# Autodesk Inventor assembly: caseBody_basePlate
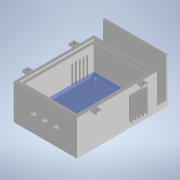
[picture p0: Inventor's stored thumbnail of the model, 180x180]
Saved by Autodesk Inventor 2022.6 (Build 266554010, 554A)
## iProperties
Created: 2025-03-20
Part Number: caseBody_basePlate
Document SubType Name: Assembly
Designer: khinm
Author: khinm
## Documents named in this file (3)
- C:\Users\khinm\Downloads\CAD\toolkit_controllerCaseDesign\caseBody_basePlate.iam
- C:\Users\khinm\Downloads\CAD\basePlate.ipt
- C:\Users\khinm\Downloads\CAD\caseBody.ipt
## Components (2 placed, 2 different names)
1. basePlate:1 — Mate:1
2. caseBody:1 — Mate:1
## Relationships (1: Mate 1)
- Mate:1: basePlate:1 ↔ caseBody:1
